# Autodesk Inventor assembly: zlozenie_palec_lewy
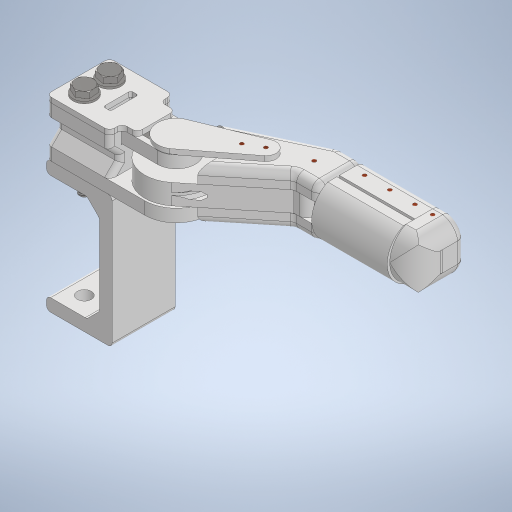
[picture p0: Inventor's stored thumbnail of the model, 512x512]
Saved by Autodesk Inventor 2024.2 (Build 282272000, 272)
## iProperties
Created: 2024-01-20
Part Number: zlozenie_palec_lewy
Document SubType Name: Assembly
Designer: Konrad
Author: Konrad
## Documents named in this file (21)
- D:\Inventor\magisterka\prototyp_2\zlozenie_palec_lewy.iam
- D:\Inventor\magisterka\prototyp_2\finger_rig.ipt
- D:\Inventor\magisterka\prototyp_2\holder_v2.ipt
- D:\Inventor\magisterka\prototyp_2\nit_skrecany.ipt
- D:\Inventor\magisterka\prototyp_2\opuszek.ipt
- D:\Inventor\magisterka\prototyp_2\palec1.ipt
- D:\Inventor\magisterka\prototyp_2\palec2.ipt
- D:\Inventor\magisterka\prototyp_2\palec3.ipt
- D:\Inventor\magisterka\prototyp_2\paliczek_v2.ipt
- D:\Inventor\magisterka\prototyp_2\pokrywka.ipt
- D:\Inventor\magisterka\prototyp_2\potentiometr_case.ipt
- D:\Inventor\magisterka\prototyp_2\pret20mm.ipt
- D:\Inventor\magisterka\prototyp_2\pret22mm.ipt
- D:\Inventor\magisterka\prototyp_2\tuleja.ipt
- D:\Inventor\magisterka\prototyp_2\tweaker.ipt
- D:\Inventor\magisterka\prototyp_2\wciskacz_v2.ipt
- C:\Users\Konrad\Documents\Inventor\Content Center Files\R2024\pl-PL\DIN 125-1  A\DIN 125 - A 4,3.ipt
- C:\Users\Konrad\Documents\Inventor\Content Center Files\R2024\pl-PL\DIN EN 24 017\ISO 4017 - M4 x 35DIN EN.ipt
- C:\Users\Konrad\Documents\Inventor\Content Center Files\R2024\pl-PL\DIN 934\DIN 934 - M4 x 0,7.ipt
- D:\Inventor\magisterka\prototyp_2\potencjometr.ipt
- D:\Inventor\magisterka\prototyp_2\czujnik_nacisku.ipt
## Components (31 placed, 20 different names)
1. finger_rig:1 — Zestawiające:1, Zestawiające:2, Zestawiające:3, Zestawiające:52, Zestawiające:54, Zestawiające:60
2. holder_v2:1 — Zestawiające:1, Zestawiające:2, Zestawiające:3, Zestawiające:28, Zestawiające:29, Zestawiające:30, Zestawiające:31, Zestawiające:32, Zestawiające:33, Zestawiające:34, Zestawiające:35, Zestawiające:61, Zestawiające:64
3. nit_skrecany:1 — Zestawiające:5, Zestawiające:6, Zestawiające:7, Zestawiające:10, Zestawiające:34, Zestawiające:35, Zestawiające:63
4. opuszek:1 — Zestawiające:46, Równoległe:13, Zestawiające:73, Zestawiające:75, Zestawiające:76
5. palec1:1 — Zestawiające:62, Zestawiające:63, Zestawiające:65, Zestawiające:66, Zestawiające:67, Zestawiające:68, Zestawiające:71, Zestawiające:73, Zestawiające:74, Zestawiające:78, Zestawiające:79, Zestawiające:82, Zestawiające:83, Zestawiające:86
6. palec2:1 — Zestawiające:15, Zestawiające:16, Zestawiające:41, Zestawiające:78, Zestawiające:84, Równoległe:16, Równoległe:17
7. palec3:1 — Zestawiające:15, Zestawiające:16, Zestawiające:79, Zestawiające:80, Zestawiające:81, Równoległe:18
8. paliczek_v2:1 — Równoległe:15, Zestawiające:68, Zestawiające:69, Zestawiające:70
9. pokrywka:1 — Zestawiające:31, Zestawiające:32, Zestawiające:33, Zestawiające:47, Zestawiające:48, Zestawiające:49, Zestawiające:50, Zestawiające:51, Zestawiające:53
10. potentiometr_case:1 — Zestawiające:28, Zestawiające:29, Zestawiające:30, Zestawiające:56, Zestawiające:57, Zestawiające:77
11. pret20mm:1 — Zestawiające:43, Równoległe:8
12. tuleja:1 — Zestawiające:5, Zestawiające:55
13. tweaker:1 — Zestawiające:77, Zestawiające:85, Równoległe:19
14. wciskacz_v2:1 — Równoległe:5, Zestawiające:72, Zestawiające:76
15. DIN 125-1 A A 4,3:1 — Zestawiające:6, Zestawiające:10
16. DIN 125-1 A A 4,3:2 — Zestawiające:7, Zestawiające:62, Zestawiające:64
17. paliczek_v2:2 — Równoległe:5, Zestawiające:42, Zestawiające:43, Zestawiające:44, Równoległe:7, Równoległe:8, Równoległe:9, Zestawiające:59, Zestawiające:65, Zestawiające:75
18. pret20mm:2 — Zestawiające:44, Równoległe:7, Zestawiające:66, Zestawiające:70
19. pret20mm:3 — Zestawiające:42, Równoległe:9, Zestawiające:67, Zestawiające:69
20. pret20mm:4 — Zestawiające:41, Zestawiające:82, Równoległe:18
21. pret22mm:2 — Zestawiające:81, Zestawiające:83, Równoległe:16, Równoległe:19
22. pret22mm:3 — Zestawiające:80, Zestawiające:84, Równoległe:17, Zestawiające:85
23. pret20mm:5 — Zestawiające:46, Równoległe:13, Zestawiające:74
24. DIN 125-1 A A 4,3:3 — Zestawiające:47, Zestawiające:48, Wstawiające:1
25. DIN EN 24017 M4 x 35:1 — Wstawiające:1
26. DIN 934 - zastąpiona przez DIN EN 24032/28673/28674 M4:1 — Zestawiające:51, Zestawiające:52
27. DIN 125-1 A A 4,3:4 — Zestawiające:49, Zestawiające:50, Wstawiające:2
28. DIN EN 24017 M4 x 35:2 — Wstawiające:2
29. DIN 934 - zastąpiona przez DIN EN 24032/28673/28674 M4:2 — Zestawiające:53, Zestawiające:54
30. potencjometr:1 — Zestawiające:55, Zestawiające:56, Zestawiające:57
31. czujnik_nacisku:1 — Równoległe:15, Zestawiające:59, Zestawiające:71, Zestawiające:72
## Relationships (73: Mate 61, Flush 10, Insert 2)
- Zestawiające:1 [Mate]: finger_rig:1 ↔ holder_v2:1
- Zestawiające:2 [Mate]: finger_rig:1 ↔ holder_v2:1
- Zestawiające:3 [Mate]: finger_rig:1 ↔ holder_v2:1
- Zestawiające:5 [Mate]: nit_skrecany:1 ↔ tuleja:1
- Zestawiające:6 [Mate]: nit_skrecany:1 ↔ DIN 125-1 A A 4,3:1
- Zestawiające:7 [Mate]: nit_skrecany:1 ↔ DIN 125-1 A A 4,3:2
- Zestawiające:10 [Mate]: nit_skrecany:1 ↔ DIN 125-1 A A 4,3:1
- Zestawiające:15 [Mate]: palec2:1 ↔ palec3:1
- Zestawiające:16 [Mate]: palec2:1 ↔ palec3:1
- Równoległe:5 [Flush]: wciskacz_v2:1 ↔ paliczek_v2:2
- Zestawiające:28 [Mate]: holder_v2:1 ↔ potentiometr_case:1
- Zestawiające:29 [Mate]: holder_v2:1 ↔ potentiometr_case:1
- Zestawiające:30 [Mate]: holder_v2:1 ↔ potentiometr_case:1
- Zestawiające:31 [Mate]: holder_v2:1 ↔ pokrywka:1
- Zestawiające:32 [Mate]: holder_v2:1 ↔ pokrywka:1
- Zestawiające:33 [Mate]: holder_v2:1 ↔ pokrywka:1
- Zestawiające:34 [Mate]: holder_v2:1 ↔ nit_skrecany:1
- Zestawiające:35 [Mate]: holder_v2:1 ↔ nit_skrecany:1
- Zestawiające:41 [Mate]: palec2:1 ↔ pret20mm:4
- Zestawiające:42 [Mate]: paliczek_v2:2 ↔ pret20mm:3
- Zestawiające:43 [Mate]: pret20mm:1 ↔ paliczek_v2:2
- Zestawiające:44 [Mate]: paliczek_v2:2 ↔ pret20mm:2
- Równoległe:7 [Flush]: paliczek_v2:2 ↔ pret20mm:2
- Równoległe:8 [Flush]: pret20mm:1 ↔ paliczek_v2:2
- Równoległe:9 [Flush]: paliczek_v2:2 ↔ pret20mm:3
- Zestawiające:46 [Mate]: opuszek:1 ↔ pret20mm:5
- Równoległe:13 [Flush]: opuszek:1 ↔ pret20mm:5
- Zestawiające:47 [Mate]: pokrywka:1 ↔ DIN 125-1 A A 4,3:3
- Zestawiające:48 [Mate]: pokrywka:1 ↔ DIN 125-1 A A 4,3:3
- Zestawiające:49 [Mate]: pokrywka:1 ↔ DIN 125-1 A A 4,3:4
- Zestawiające:50 [Mate]: pokrywka:1 ↔ DIN 125-1 A A 4,3:4
- Wstawiające:1 [Insert]: DIN 125-1 A A 4,3:3 ↔ DIN EN 24017 M4 x 35:1
- Wstawiające:2 [Insert]: DIN 125-1 A A 4,3:4 ↔ DIN EN 24017 M4 x 35:2
- Zestawiające:51 [Mate]: pokrywka:1 ↔ DIN 934 - zastąpiona przez DIN EN 24032/28673/28674 M4:1
- Zestawiające:52 [Mate]: finger_rig:1 ↔ DIN 934 - zastąpiona przez DIN EN 24032/28673/28674 M4:1
- Zestawiające:53 [Mate]: pokrywka:1 ↔ DIN 934 - zastąpiona przez DIN EN 24032/28673/28674 M4:2
- Zestawiające:54 [Mate]: finger_rig:1 ↔ DIN 934 - zastąpiona przez DIN EN 24032/28673/28674 M4:2
- Zestawiające:55 [Mate]: tuleja:1 ↔ potencjometr:1
- Zestawiające:56 [Mate]: potentiometr_case:1 ↔ potencjometr:1
- Zestawiające:57 [Mate]: potentiometr_case:1 ↔ potencjometr:1
- Równoległe:15 [Flush]: paliczek_v2:1 ↔ czujnik_nacisku:1
- Zestawiające:59 [Mate]: paliczek_v2:2 ↔ czujnik_nacisku:1
- Zestawiające:60 [Mate]: finger_rig:1
- Zestawiające:61 [Mate]: holder_v2:1
- Zestawiające:62 [Mate]: palec1:1 ↔ DIN 125-1 A A 4,3:2
- Zestawiające:63 [Mate]: nit_skrecany:1 ↔ palec1:1
- Zestawiające:64 [Mate]: holder_v2:1 ↔ DIN 125-1 A A 4,3:2
- Zestawiające:65 [Mate]: palec1:1 ↔ paliczek_v2:2
- Zestawiające:66 [Mate]: palec1:1 ↔ pret20mm:2
- Zestawiające:67 [Mate]: palec1:1 ↔ pret20mm:3
- Zestawiające:68 [Mate]: palec1:1 ↔ paliczek_v2:1
- Zestawiające:69 [Mate]: paliczek_v2:1 ↔ pret20mm:3
- Zestawiające:70 [Mate]: paliczek_v2:1 ↔ pret20mm:2
- Zestawiające:71 [Mate]: palec1:1 ↔ czujnik_nacisku:1
- Zestawiające:72 [Mate]: wciskacz_v2:1 ↔ czujnik_nacisku:1
- Zestawiające:73 [Mate]: opuszek:1 ↔ palec1:1
- Zestawiające:74 [Mate]: palec1:1 ↔ pret20mm:5
- Zestawiające:75 [Mate]: opuszek:1 ↔ paliczek_v2:2
- Zestawiające:76 [Mate]: opuszek:1 ↔ wciskacz_v2:1
- Zestawiające:77 [Mate]: potentiometr_case:1 ↔ tweaker:1
- Zestawiające:78 [Mate]: palec1:1 ↔ palec2:1
- Zestawiające:79 [Mate]: palec1:1 ↔ palec3:1
- Zestawiające:80 [Mate]: palec3:1 ↔ pret22mm:3
- Zestawiające:81 [Mate]: palec3:1 ↔ pret22mm:2
- Zestawiające:82 [Mate]: palec1:1 ↔ pret20mm:4
- Zestawiające:83 [Mate]: palec1:1 ↔ pret22mm:2
- Zestawiające:84 [Mate]: palec2:1 ↔ pret22mm:3
- Równoległe:16 [Flush]: palec2:1 ↔ pret22mm:2
- Równoległe:17 [Flush]: palec2:1 ↔ pret22mm:3
- Równoległe:18 [Flush]: palec3:1 ↔ pret20mm:4
- Zestawiające:85 [Mate]: tweaker:1 ↔ pret22mm:3
- Równoległe:19 [Flush]: tweaker:1 ↔ pret22mm:2
- Zestawiające:86 [Mate]: palec1:1
